# Autodesk Inventor assembly: Drivebase
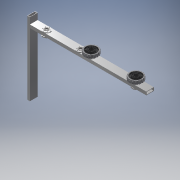
[picture p0: Inventor's stored thumbnail of the model, 180x180]
Saved by Autodesk Inventor 2019.4 (Build 234330000, 330)
## iProperties
Created: 2020-01-05
Part Number: Drivebase
Document SubType Name: Assembly
Designer: Mark
Author: Mark
## Documents named in this file (5)
- C:\Users\Mark\Desktop\7738 Helion Engineering\7738-2020\CAD\Drivebase.iam
- C:\Users\Mark\Desktop\7738 Helion Engineering\7738-2020\CAD\Main Extrusion.ipt
- C:\Users\Mark\Desktop\7738 Helion Engineering\7738-2020\CAD\Back Extrusion.ipt
- C:\Users\Mark\Desktop\7738 Helion Engineering\7738-2020\CAD\Bearing Block Assembly.iam
- C:\Users\Mark\Desktop\7738 Helion Engineering\7738-2020\CAD\4_VersaWheel_DT_217-3197.ipt
## Components (10 placed, 4 different names)
1. Main Extrusion:1 — Mate:1, Flush:1, Flush:2, Mate:2, Mate:3, Mate:4, Mate:5, Mate:6, Mate:7, Mate:8, Mate:9, Mate:10, Mate:11, Mate:12, Mate:13, Mate:14, Mate:15, Mate:16, Mate:17, Mate:18, Mate:19
2. Back Extrusion:1 — Mate:1, Flush:1, Flush:2
3. Bearing Block Assembly:1 [sub-assembly] — Mate:2, Mate:3, Mate:4
4. Bearing Block Assembly:2 [sub-assembly] — Mate:5, Mate:6, Mate:7
5. Bearing Block Assembly:3 [sub-assembly] — Mate:11, Mate:12, Mate:13
6. Bearing Block Assembly:4 [sub-assembly] — Mate:8, Mate:9, Mate:10, Mate:20, Mate:21
7. Bearing Block Assembly:5 [sub-assembly] — Mate:14, Mate:15, Mate:16
8. Bearing Block Assembly:6 [sub-assembly] — Mate:17, Mate:18, Mate:19, Mate:22, Mate:23
9. 4_VersaWheel_DT_217-3197:1 — Mate:22, Mate:23
10. 4_VersaWheel_DT_217-3197:2 — Mate:20, Mate:21
## Relationships (25: Mate 23, Flush 2)
- Mate:1: Main Extrusion:1 ↔ Back Extrusion:1
- Flush:1: Main Extrusion:1 ↔ Back Extrusion:1
- Flush:2 (-50 mm): Main Extrusion:1 ↔ Back Extrusion:1
- Mate:2: Main Extrusion:1 ↔ Bearing Block Assembly:1
- Mate:3: Main Extrusion:1 ↔ Bearing Block Assembly:1
- Mate:4: Main Extrusion:1 ↔ Bearing Block Assembly:1
- Mate:5: Main Extrusion:1 ↔ Bearing Block Assembly:2
- Mate:6: Main Extrusion:1 ↔ Bearing Block Assembly:2
- Mate:7: Main Extrusion:1 ↔ Bearing Block Assembly:2
- Mate:8: Main Extrusion:1 ↔ Bearing Block Assembly:4
- Mate:9: Main Extrusion:1 ↔ Bearing Block Assembly:4
- Mate:10: Main Extrusion:1 ↔ Bearing Block Assembly:4
- Mate:11: Main Extrusion:1 ↔ Bearing Block Assembly:3
- Mate:12: Main Extrusion:1 ↔ Bearing Block Assembly:3
- Mate:13: Main Extrusion:1 ↔ Bearing Block Assembly:3
- Mate:14: Main Extrusion:1 ↔ Bearing Block Assembly:5
- Mate:15: Main Extrusion:1 ↔ Bearing Block Assembly:5
- Mate:16: Main Extrusion:1 ↔ Bearing Block Assembly:5
- Mate:17: Main Extrusion:1 ↔ Bearing Block Assembly:6
- Mate:18: Main Extrusion:1 ↔ Bearing Block Assembly:6
- Mate:19: Main Extrusion:1 ↔ Bearing Block Assembly:6
- Mate:20: Bearing Block Assembly:4 ↔ 4_VersaWheel_DT_217-3197:2
- Mate:21 (7 mm): Bearing Block Assembly:4 ↔ 4_VersaWheel_DT_217-3197:2
- Mate:22: Bearing Block Assembly:6 ↔ 4_VersaWheel_DT_217-3197:1
- Mate:23 (7 mm): Bearing Block Assembly:6 ↔ 4_VersaWheel_DT_217-3197:1
